# Autodesk Inventor assembly: Joint_2
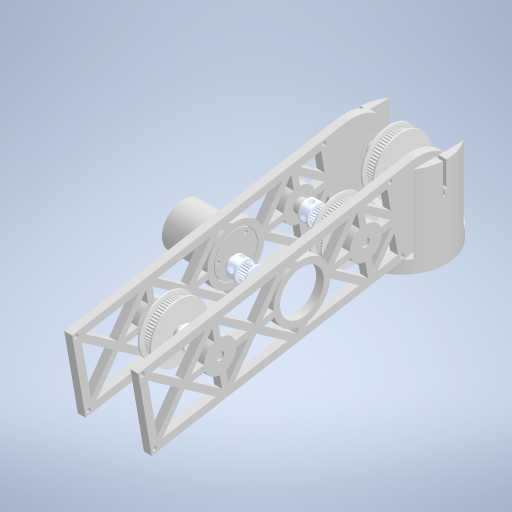
[picture p0: Inventor's stored thumbnail of the model, 512x512]
Saved by Autodesk Inventor 2023 (Build 270158030, 158C)
## iProperties
Created: 2022-06-17
Part Number: Joint_2
Document SubType Name: Assembly
Designer: Mlees
Author: Mlees
## Documents named in this file (13)
- E:\504Engineering\Project_0000\Mechanical\Joint_2\Joint_2.iam
- E:\504Engineering\Project_0000\Mechanical\Joint_2\Aluminum_Rod.ipt
- E:\504Engineering\Project_0000\Mechanical\Joint_2\Bearing.ipt
- E:\504Engineering\Project_0000\Mechanical\Joint_2\Motor.ipt
- E:\504Engineering\Project_0000\Mechanical\Joint_2\Side_Piece.ipt
- E:\504Engineering\Project_0000\Mechanical\downloaded_parts\gt2-pulley-6.snapshot.2\GT2 Timing Pulley.ipt
- E:\504Engineering\Project_0000\Mechanical\downloaded_parts\gt2-60-teeth-pulley-1.snapshot.4\GT2 60 teeth pulley.ipt
- E:\504Engineering\Project_0000\Mechanical\Joint_2\Spacer_5mm_6mm.ipt
- E:\504Engineering\Project_0000\Mechanical\Joint_2\Spacer_5mm_3mm.ipt
- E:\504Engineering\Project_0000\Mechanical\Joint_2\Spacer_5mm_3-5mm.ipt
- E:\504Engineering\Project_0000\Mechanical\Joint_2\Spacer_5mm_22mm.ipt
- E:\504Engineering\Project_0000\Mechanical\Joint_2\Aluminum_Rod_70mm.ipt
- E:\504Engineering\Project_0000\Mechanical\Joint_2\Base.ipt
## Components (26 placed, 12 different names)
1. Aluminum_Rod:1 — Mate:6, Flush:2, Mate:15, Mate:16, Mate:19, Mate:21, Mate:25
2. Bearing:1 — Mate:1, Mate:2, Mate:6, Flush:2, Mate:17
3. Motor:1 — Mate:29, Mate:30, Rigid:1
4. Side_Piece:1 — Mate:1, Mate:2, Mate:3, Mate:4, Mate:43, Flush:5, Rigid:1
5. Bearing:2 — Mate:3, Mate:4, Mate:5, Flush:1, Mate:36
6. Aluminum_Rod:2 — Mate:5, Flush:1, Mate:9, Mate:11, Mate:13, Mate:23, Mate:35, Mate:39
7. GT2 Timing Pulley:1 — Mate:9, Mate:38, Mate:40, Rotation:2, Rotation:3
8. GT2 Timing Pulley:2 — Mate:16, Mate:18, Mate:20, Rotation:4, Rotation:5
9. GT2 60 teeth pulley:1 — Mate:11, Mate:37, Mate:41, Rotation:1, Rotation:3
10. GT2 60 teeth pulley:2 — Mate:19, Mate:20, Mate:22, Rotation:2, Rotation:4
11. Spacer_5mm_6mm:2 — Mate:13, Mate:24, Mate:38
12. Spacer_5mm_6mm:3 — Mate:15, Mate:17, Mate:18
13. Spacer_5mm_6mm:4 — Mate:21, Mate:22, Mate:26
14. Bearing:3 — Mate:23, Mate:24, Mate:31
15. Bearing:4 — Mate:25, Mate:26, Mate:32, Flush:3
16. GT2 Timing Pulley:3 — Mate:29, Mate:30, Rotation:1
17. Side_Piece:2 — Mate:31, Mate:32, Flush:3, Mate:42, Flush:4, Mate:51
18. Spacer_5mm_3mm:1 — Mate:35, Mate:36, Mate:37
19. Spacer_5mm_3-5mm:1 — Mate:39, Mate:40, Mate:41
20. Bearing:5 — Mate:42, Flush:4, Mate:48, Mate:50
21. Bearing:6 — Mate:43, Flush:5, Mate:44, Mate:45
22. Spacer_5mm_6mm:5 — Mate:44, Mate:45, Mate:46, Mate:47
23. GT2 60 teeth pulley:3 — Mate:46, Mate:47, Mate:49, Rotation:5
24. Spacer_5mm_22mm:1 — Mate:48, Mate:49
25. Aluminum_Rod_70mm:1 — Mate:50, Mate:52, Mate:53, Mate:54, Mate:55
26. Base:1 — Mate:51, Mate:52, Mate:53, Mate:54, Mate:55
## Relationships (57: Mate 46, Flush 5, RelateRotation 5, WeldJoint 1)
- Mate:1: Bearing:1 ↔ Side_Piece:1
- Mate:2: Bearing:1 ↔ Side_Piece:1
- Mate:3: Side_Piece:1 ↔ Bearing:2
- Mate:4: Side_Piece:1 ↔ Bearing:2
- Mate:5: Bearing:2 ↔ Aluminum_Rod:2
- Mate:6: Aluminum_Rod:1 ↔ Bearing:1
- Flush:1: Bearing:2 ↔ Aluminum_Rod:2
- Flush:2: Aluminum_Rod:1 ↔ Bearing:1
- Mate:9: Aluminum_Rod:2 ↔ GT2 Timing Pulley:1
- Mate:11: Aluminum_Rod:2 ↔ GT2 60 teeth pulley:1
- Mate:13: Aluminum_Rod:2 ↔ Spacer_5mm_6mm:2
- Mate:15: Aluminum_Rod:1 ↔ Spacer_5mm_6mm:3
- Mate:16: Aluminum_Rod:1 ↔ GT2 Timing Pulley:2
- Mate:17: Bearing:1 ↔ Spacer_5mm_6mm:3
- Mate:18: GT2 Timing Pulley:2 ↔ Spacer_5mm_6mm:3
- Mate:19: Aluminum_Rod:1 ↔ GT2 60 teeth pulley:2
- Mate:20: GT2 Timing Pulley:2 ↔ GT2 60 teeth pulley:2
- Mate:21: Aluminum_Rod:1 ↔ Spacer_5mm_6mm:4
- Mate:22: GT2 60 teeth pulley:2 ↔ Spacer_5mm_6mm:4
- Mate:23: Aluminum_Rod:2 ↔ Bearing:3
- Mate:24: Spacer_5mm_6mm:2 ↔ Bearing:3
- Mate:25: Aluminum_Rod:1 ↔ Bearing:4
- Mate:26: Spacer_5mm_6mm:4 ↔ Bearing:4
- Mate:29: Motor:1 ↔ GT2 Timing Pulley:3
- Mate:30: Motor:1 ↔ GT2 Timing Pulley:3
- Mate:31: Bearing:3 ↔ Side_Piece:2
- Mate:32: Bearing:4 ↔ Side_Piece:2
- Flush:3: Bearing:4 ↔ Side_Piece:2
- Mate:35: Aluminum_Rod:2 ↔ Spacer_5mm_3mm:1
- Mate:36: Bearing:2 ↔ Spacer_5mm_3mm:1
- Mate:37: GT2 60 teeth pulley:1 ↔ Spacer_5mm_3mm:1
- Mate:38: GT2 Timing Pulley:1 ↔ Spacer_5mm_6mm:2
- Mate:39: Aluminum_Rod:2 ↔ Spacer_5mm_3-5mm:1
- Mate:40: GT2 Timing Pulley:1 ↔ Spacer_5mm_3-5mm:1
- Mate:41: GT2 60 teeth pulley:1 ↔ Spacer_5mm_3-5mm:1
- Mate:42: Side_Piece:2 ↔ Bearing:5
- Flush:4: Side_Piece:2 ↔ Bearing:5
- Mate:43: Side_Piece:1 ↔ Bearing:6
- Flush:5: Side_Piece:1 ↔ Bearing:6
- Mate:44: Bearing:6 ↔ Spacer_5mm_6mm:5
- Mate:45: Bearing:6 ↔ Spacer_5mm_6mm:5
- Mate:46: Spacer_5mm_6mm:5 ↔ GT2 60 teeth pulley:3
- Mate:47: Spacer_5mm_6mm:5 ↔ GT2 60 teeth pulley:3
- Mate:48: Bearing:5 ↔ Spacer_5mm_22mm:1
- Mate:49: GT2 60 teeth pulley:3 ↔ Spacer_5mm_22mm:1
- Mate:50: Bearing:5 ↔ Aluminum_Rod_70mm:1
- Mate:51: Side_Piece:2 ↔ Base:1
- Mate:52: Aluminum_Rod_70mm:1 ↔ Base:1
- Mate:53: Aluminum_Rod_70mm:1 ↔ Base:1
- Mate:54: Aluminum_Rod_70mm:1 ↔ Base:1
- Mate:55: Aluminum_Rod_70mm:1 ↔ Base:1
- Rotation:1 [RelateRotation] (0.3333 ul): GT2 60 teeth pulley:1 ↔ GT2 Timing Pulley:3
- Rotation:2 [RelateRotation] (0.3333 ul): GT2 Timing Pulley:1 ↔ GT2 60 teeth pulley:2
- Rigid:1 [WeldJoint]: Motor:1 ↔ Side_Piece:1
- Rotation:3 [RelateRotation] (1 ul): GT2 Timing Pulley:1 ↔ GT2 60 teeth pulley:1
- Rotation:4 [RelateRotation] (1 ul): GT2 Timing Pulley:2 ↔ GT2 60 teeth pulley:2
- Rotation:5 [RelateRotation] (0.3333 ul): GT2 Timing Pulley:2 ↔ GT2 60 teeth pulley:3
